# Autodesk Inventor assembly: ADSK-MH-10019
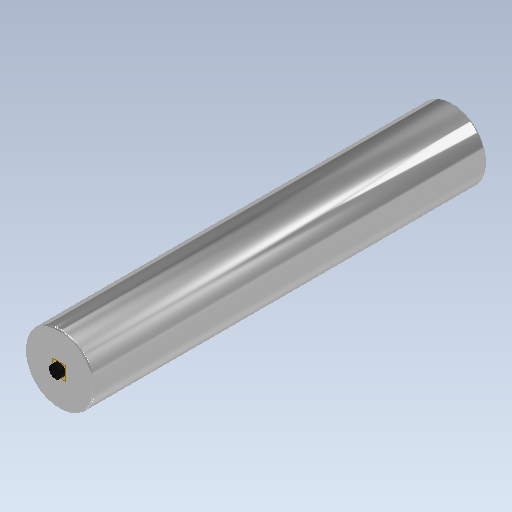
[picture p0: Inventor's stored thumbnail of the model, 512x512]
Saved by Autodesk Inventor 2020.2 (Build 242310000, 310)
## iProperties
Created: 2008-03-10
Part Number: ADSK-MH-10019
Document SubType Name: Assembly
Designer: R.O'mahony
Description: Roller Assembly
Engineer: Demir Ali
Checked By: Demir Ali
Company: Autodesk Ltd
Author: R.O'mahony
Keywords: Roller Conveyor
Revision Number: A
## Documents named in this file (3)
- C:\Users\peter\source\repos\InventorDA-FLC\Dataset\Discharge Conveyor\ADSK-MH-10019.iam
- C:\Users\peter\source\repos\InventorDA-FLC\Dataset\Discharge Conveyor\ADSK-MH-10022.ipt
- C:\Users\peter\source\repos\InventorDA-FLC\Dataset\Discharge Conveyor\ADSK-MH-10023.ipt
## Components (2 placed, 2 different names)
1. Top_Roller_bar — Flush:1
2. Top_Roller — Flush:1
## Relationships (1: Flush 1)
- Flush:1: Top_Roller_bar ↔ Top_Roller
